# Autodesk Inventor assembly: Foot
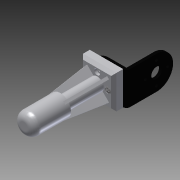
[picture p0: Inventor's stored thumbnail of the model, 180x180]
Saved by Autodesk Inventor 2015 (Build 190159000, 159)
## iProperties
Created: 2015-05-22
Part Number: Foot
Document SubType Name: Assembly
Designer: Quinn
Author: Quinn
## Documents named in this file (4)
- C:\Users\Quinn\Desktop\3DCNC Design\InventorModels\Assemblies\Foot.iam
- C:\Users\Quinn\Desktop\3DCNC Design\InventorModels\Plastics\QuadrupedFoot.ipt
- C:\Users\Quinn\Desktop\3DCNC Design\InventorModels\Metal\Brackets\asb-06-LTab.ipt
- C:\Users\Quinn\Desktop\3DCNC Design\InventorModels\Assemblies\Foot\Design Accelerator\Bolted Connection1.iam
## Components (3 placed, 3 different names)
1. QuadrupedFoot:1 — Insert:1, Mate:1, Mate:2
2. asb-06-LTab:1 — Insert:1
3. Bolted Connection:1 [sub-assembly] — Mate:1, Mate:2
## Relationships (3: Mate 2, Insert 1)
- Insert:1: QuadrupedFoot:1 ↔ asb-06-LTab:1
- Mate:1: QuadrupedFoot:1 ↔ Bolted Connection:1
- Mate:2: QuadrupedFoot:1 ↔ Bolted Connection:1
